# Autodesk Inventor assembly: 1st arm draft
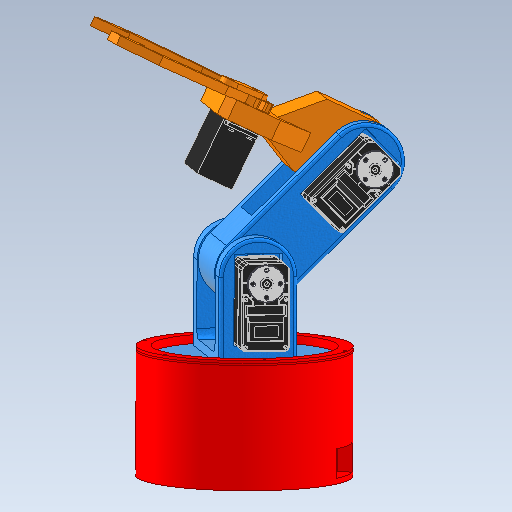
[picture p0: Inventor's stored thumbnail of the model, 512x512]
Saved by Autodesk Inventor 2026 (Build 300175050, 175E)
## iProperties
Created: 2026-02-04
Part Number: 1st arm draft
Document SubType Name: Assembly
Designer: morga
Author: morga
## Documents named in this file (10)
- D:\MechGroupProject\1st arm draft.iam
- D:\MechGroupProject\ShoulderJoint.ipt
- D:\MechGroupProject\BicepJoint.ipt
- D:\MechGroupProject\ST3215\ST3215\ST3215.ipt
- D:\MechGroupProject\Arm\Arm\Arm.ipt
- D:\MechGroupProject\Arm 2\Arm 2\Arm 2.ipt
- D:\MechGroupProject\basecap.ipt
- D:\MechGroupProject\forearmJoint2.ipt
- D:\MechGroupProject\Futaba FP-S28\servo motor\servo motor\servo motor.ipt
- D:\MechGroupProject\base.ipt
## Components (10 placed, 9 different names)
1. ShoulderJoint:1 — Mate:3, Mate:4, Mate:5, Insert:33, Insert:34
2. BicepJoint:1 — Insert:26, Insert:27, Mate:12
3. ST3215:1 — Insert:27, Mate:12, Insert:32
4. ST3215:2 — Mate:3, Mate:4, Mate:5, Insert:26
5. Arm 2:1 — Insert:30, Mate:19
6. Arm:1 — Insert:35, Mate:19
7. forearmJoint2:1 — Insert:29, Mate:13, Mate:14, Mate:15, Mate:16, Insert:30, Insert:32
8. servo motor:1 — Insert:29, Mate:13, Mate:14, Mate:15, Mate:16, Insert:35
9. basecap:1 — Insert:34, Mate:17, Mate:18
10. base:1 — Insert:33, Mate:17, Mate:18
## Relationships (19: Mate 11, Insert 8)
- Mate:3: ShoulderJoint:1 ↔ ST3215:2
- Mate:4: ShoulderJoint:1 ↔ ST3215:2
- Mate:5: ShoulderJoint:1 ↔ ST3215:2
- Insert:26 (-4 mm): BicepJoint:1 ↔ ST3215:2
- Insert:27: BicepJoint:1 ↔ ST3215:1
- Mate:12: BicepJoint:1 ↔ ST3215:1
- Insert:29: forearmJoint2:1 ↔ servo motor:1
- Mate:13: forearmJoint2:1 ↔ servo motor:1
- Mate:14: forearmJoint2:1 ↔ servo motor:1
- Mate:15: forearmJoint2:1 ↔ servo motor:1
- Mate:16: forearmJoint2:1 ↔ servo motor:1
- Insert:30 (-5 mm): Arm 2:1 ↔ forearmJoint2:1
- Insert:32: ST3215:1 ↔ forearmJoint2:1
- Insert:33: ShoulderJoint:1 ↔ base:1
- Insert:34: ShoulderJoint:1 ↔ basecap:1
- Mate:17: basecap:1 ↔ base:1
- Mate:18: basecap:1 ↔ base:1
- Insert:35 (6 mm): Arm:1 ↔ servo motor:1
- Mate:19: Arm 2:1 ↔ Arm:1
